# Autodesk Inventor assembly: Slider_crank_mechanism
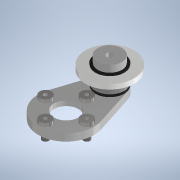
[picture p0: Inventor's stored thumbnail of the model, 180x180]
Saved by Autodesk Inventor 2020 (Build 240168000, 168)
## iProperties
Created: 2021-09-06
Part Number: Slider_crank_mechanism
Document SubType Name: Assembly
Designer: Masato Kubotera
Mass: 2.53036 g
Surface Area: 18.5815 cm^2
Volume: 1.13409 cm^3
Density: 2.23118 g/cm^3
Author: Masato Kubotera
## Documents named in this file (9)
- C:\Users\Masato\Documents\Inventor\CIT Brains_Inventor\OpenPlatform_ver3_0\LowerBody\Slider_crank\Slider_crank_mechanism.iam
- C:\Users\Masato\Documents\Inventor\CIT Brains_Inventor\OpenPlatform_ver3_0\LowerBody\Slider_crank\Slider_crank_horn.ipt
- C:\Users\Masato\Documents\Inventor\CIT Brains_Inventor\OpenPlatform_ver3_0\Ready_Made\LED-0606.ipt
- C:\Users\Masato\Documents\Inventor\CIT Brains_Inventor\OpenPlatform_ver3_0\Ready_Made\Screw\M2_6-6.ipt
- C:\Users\Masato\Documents\Inventor\CIT Brains_Inventor\OpenPlatform_ver3_0\Ready_Made\TT-1020-20.ipt
- C:\Users\Masato\Documents\Inventor\CIT Brains_Inventor\OpenPlatform_ver3_0\Ready_Made\UUW-0412-10BH.ipt
- C:\Users\Masato\Documents\Inventor\CIT Brains_Inventor\OpenPlatform_ver3_0\Ready_Made\S4-07-3W.ipt
- C:\Users\Masato\Documents\Inventor\CIT Brains_Inventor\OpenPlatform_ver3_0\Ready_Made\UUW-0612-05BH.ipt
- C:\Users\Masato\Documents\Inventor\CIT Brains_Inventor\OpenPlatform_ver3_0\Ready_Made\DBS4-7-4.ipt
## Components (11 placed, 8 different names)
1. LED-0606:1 — 挿入:23
2. M2_6-6:1 — 挿入:18
3. M2_6-6:2 — 挿入:20
4. M2_6-6:3 — 挿入:19
5. M2_6-6:4 — 挿入:21
6. TT-1020-20:1 — 挿入:27
7. Slider_crank_horn:1 — 挿入:18, 挿入:19, 挿入:20, 挿入:21, メイト:1, フラッシュ:1, メイト:2, 挿入:24, 角度:1, 挿入:25
8. UUW-0412-10BH:1 — 挿入:23, 挿入:24, 挿入:28
9. S4-07-3W:1 — 角度:1, 挿入:25
10. UUW-0612-05BH:1 — 挿入:27, 挿入:29
11. DBS4-7-4:1 — 挿入:28, 挿入:29
## Relationships (14: Insert 10, Mate 2, Flush 1, Angle 1)
- 挿入:18 [Insert]: M2_6-6:1 ↔ Slider_crank_horn:1
- 挿入:19 [Insert]: M2_6-6:3 ↔ Slider_crank_horn:1
- 挿入:20 [Insert]: M2_6-6:2 ↔ Slider_crank_horn:1
- 挿入:21 [Insert]: M2_6-6:4 ↔ Slider_crank_horn:1
- 挿入:23 [Insert]: LED-0606:1 ↔ UUW-0412-10BH:1
- メイト:1 [Mate]: Slider_crank_horn:1
- フラッシュ:1 [Flush]: Slider_crank_horn:1
- メイト:2 [Mate]: Slider_crank_horn:1
- 挿入:24 [Insert]: Slider_crank_horn:1 ↔ UUW-0412-10BH:1
- 角度:1 [Angle] (0 deg): Slider_crank_horn:1 ↔ S4-07-3W:1
- 挿入:25 [Insert]: Slider_crank_horn:1 ↔ S4-07-3W:1
- 挿入:27 [Insert]: TT-1020-20:1 ↔ UUW-0612-05BH:1
- 挿入:28 [Insert]: UUW-0412-10BH:1 ↔ DBS4-7-4:1
- 挿入:29 [Insert]: UUW-0612-05BH:1 ↔ DBS4-7-4:1
